# Autodesk Inventor assembly: Elevator
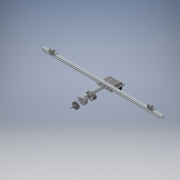
[picture p0: Inventor's stored thumbnail of the model, 180x180]
Saved by Autodesk Inventor 2017 (Build 210142000, 142)
## iProperties
Created: 2016-12-12
Part Number: Elevator
Document SubType Name: Assembly
Designer: umr
Mass: 2299.93 g
Surface Area: 5139.57 cm^2
Volume: 605.03 cm^3
Density: 3.80135 g/cm^3
Author: umr
## Documents named in this file (9)
- D:\SeniorProject\Models2\Gantry\GantryUp.iam
- D:\SeniorProject\Models2\Gantry\Tee Nut With headless screw.iam
- D:\SeniorProject\Models2\Gantry\HeaderTrack.ipt
- D:\SeniorProject\Models2\Gantry\PowerScrewNut.ipt
- D:\SeniorProject\Models2\LBent_PScrew.ipt
- D:\SeniorProject\Models2\Gantry\Tee Nut With headless screw_MIR.iam
- D:\SeniorProject\Models2\Gantry\PowerScrewNut_MIR.ipt
- D:\SeniorProject\Models2\LBent_PScrew_MIR.ipt
- D:\SeniorProject\Models2\Head\HeadSlider.iam
## Components (10 placed, 8 different names)
1. Tee Nut With headless screw:2 [sub-assembly] — Mate:79, Mate:80, Mate:85
2. HeaderTrack:1 — Mate:79, Mate:80, Mate:84, Mate:86, Flush:1, Tangent:1, Tangent:2, Mate:93, Flush:2, Mate:98
3. PowerScrewNut:1 — Mate:94, Mate:95
4. LBent_PScrew:1 — Mate:85, Mate:86, Mate:87, Flush:1, Mate:94, Mate:95
5. Tee Nut With headless screw:3 [sub-assembly] — Mate:84, Mate:87
6. Tee Nut With headless screw_MIR:1 [sub-assembly] — Mate:88, Flush:3
7. PowerScrewNut_MIR:1 — Mate:96, Mate:97
8. LBent_PScrew_MIR:1 — Mate:88, Mate:92, Mate:96, Mate:97, Flush:2, Flush:3, Flush:4
9. Tee Nut With headless screw_MIR:2 [sub-assembly] — Mate:92, Flush:4, Mate:98
10. HeadSlider:1 [sub-assembly] — Tangent:1, Tangent:2, Mate:93
## Relationships (20: Mate 14, Flush 4, Tangent 2)
- Mate:79: Tee Nut With headless screw:2 ↔ HeaderTrack:1
- Mate:80: Tee Nut With headless screw:2 ↔ HeaderTrack:1
- Mate:84: HeaderTrack:1 ↔ Tee Nut With headless screw:3
- Mate:85: Tee Nut With headless screw:2 ↔ LBent_PScrew:1
- Mate:86: HeaderTrack:1 ↔ LBent_PScrew:1
- Mate:87: LBent_PScrew:1 ↔ Tee Nut With headless screw:3
- Flush:1 (99.35 mm): HeaderTrack:1 ↔ LBent_PScrew:1
- Mate:88: Tee Nut With headless screw_MIR:1 ↔ LBent_PScrew_MIR:1
- Mate:92: LBent_PScrew_MIR:1 ↔ Tee Nut With headless screw_MIR:2
- Tangent:1: HeaderTrack:1 ↔ HeadSlider:1
- Tangent:2: HeaderTrack:1 ↔ HeadSlider:1
- Mate:93: HeaderTrack:1 ↔ HeadSlider:1
- Mate:94: PowerScrewNut:1 ↔ LBent_PScrew:1
- Mate:95: PowerScrewNut:1 ↔ LBent_PScrew:1
- Mate:96: PowerScrewNut_MIR:1 ↔ LBent_PScrew_MIR:1
- Mate:97: PowerScrewNut_MIR:1 ↔ LBent_PScrew_MIR:1
- Flush:2 (99.35 mm): HeaderTrack:1 ↔ LBent_PScrew_MIR:1
- Flush:3: Tee Nut With headless screw_MIR:1 ↔ LBent_PScrew_MIR:1
- Flush:4: LBent_PScrew_MIR:1 ↔ Tee Nut With headless screw_MIR:2
- Mate:98: HeaderTrack:1 ↔ Tee Nut With headless screw_MIR:2
